# Autodesk Inventor assembly: Skateboard Box
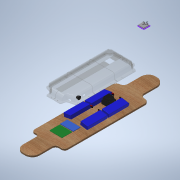
[picture p0: Inventor's stored thumbnail of the model, 180x180]
Saved by Autodesk Inventor 2020 (Build 240168000, 168)
## iProperties
Created: 2019-01-10
Part Number: Skateboard Box
Document SubType Name: Assembly
Designer: LSabe
Author: LSabe
## Documents named in this file (15)
- C:\Users\Luke\OneDrive\Desktop\Luke's stuff\Electric Skateboard\Electric_Skateboard V.2\Skateboard Files\Skateboard Box Files\Skateboard Box V2.iam
- C:\Users\Luke\OneDrive\Desktop\Luke's stuff\Electric Skateboard\Electric_Skateboard V.2\Skateboard Files\Skateboard Box Files\ESC.ipt
- C:\Users\LSabe\OneDrive\Documents\Inventor\Content Center Files\R2017\en-US\ANSI B18.6.3(03)\ANSI B18.6.3 - 10-32 UNF - 0.75(14).ipt
- C:\Users\Luke\OneDrive\Desktop\Luke's stuff\Electric Skateboard\Electric_Skateboard V.2\Skateboard Files\Skateboard Box Files\Battery.ipt
- C:\Users\Luke\OneDrive\Desktop\Luke's stuff\Electric Skateboard\Electric_Skateboard V.2\Skateboard Files\Skateboard Box Files\Lipo Charger Circuit.ipt
- C:\Users\Luke\OneDrive\Desktop\Luke's stuff\Electric Skateboard\Electric_Skateboard V.2\Skateboard Files\Skateboard Box Files\Receiver PCB.ipt
- C:\Users\Luke\OneDrive\Desktop\Luke's stuff\Electric Skateboard\Electric_Skateboard V.2\Skateboard Files\Skateboard Box Files\Power Switch.ipt
- C:\Users\Luke\OneDrive\Desktop\Luke's stuff\Electric Skateboard\Electric_Skateboard V.2\Skateboard Files\Skateboard Box Files\Skateboard Deck.ipt
- C:\Users\Luke\OneDrive\Desktop\Luke's stuff\Electric Skateboard\Electric_Skateboard V.2\Skateboard Files\Skateboard Box Files\Skateboard Box Back V2 a.ipt
- C:\Users\Luke\OneDrive\Desktop\Luke's stuff\Electric Skateboard\Electric_Skateboard V.2\Skateboard Files\Skateboard Box Files\Skateboard Box Back V2 b.ipt
- C:\Users\Luke\OneDrive\Desktop\Luke's stuff\Electric Skateboard\Electric_Skateboard V.2\Skateboard Files\Skateboard Box Files\Skateboard Box Front V2 a.ipt
- C:\Users\Luke\OneDrive\Desktop\Luke's stuff\Electric Skateboard\Electric_Skateboard V.2\Skateboard Files\Skateboard Box Files\Skateboard Box Front V2 b.ipt
- C:\Users\Luke\OneDrive\Desktop\Luke's stuff\Electric Skateboard\Electric_Skateboard V.2\Skateboard Files\Skateboard Box Files\Skateboard Box Middle V2 a.ipt
- C:\Users\Luke\OneDrive\Desktop\Luke's stuff\Electric Skateboard\Electric_Skateboard V.2\Skateboard Files\Skateboard Box Files\Skateboard Box Middle V2 b.ipt
- C:\Users\Luke\OneDrive\Desktop\Luke's stuff\Electric Skateboard\Electric_Skateboard V.2\Skateboard Files\Skateboard Box Files\Plug.ipt
## Components (34 placed, 14 different names)
1. ESC:1 — Mate:16, Mate:20
2. Receiver PCB:1 — Mate:15, Mate:17
3. Battery:1 — Mate:13, Flush:2, Flush:3
4. Battery:2 — Mate:14, Flush:2, Flush:4
5. Battery:3 — Mate:11, Flush:1, Flush:4
6. Battery:4 — Mate:12, Flush:1, Flush:3
7. Power Switch:1 — Mate:52, Mate:53
8. Skateboard Deck:1 — Mate:11, Mate:12, Mate:13, Mate:14, Mate:15, Mate:16, Mate:17, Mate:20, Mate:21, Mate:45, Mate:46, Flush:8, Flush:9, Mate:47, Mate:48, Flush:10, Mate:49
9. Lipo Charger Circuit:1 — Mate:21, Mate:45
10. Skateboard Box Back V2 a:1 — Flush:5, Flush:10, Flush:11, Flush:15, Mate:50, Mate:58, Mate:59, Mate:72, Mate:73
11. Skateboard Box Back V2 b:1 — Flush:5, Mate:48, Flush:11, Mate:64, Mate:65, Mate:68, Mate:69
12. Skateboard Box Front V2 a:1 — Flush:7, Flush:8, Flush:13, Flush:14, Mate:51, Mate:52, Mate:53, Mate:54, Mate:55, Mate:70, Mate:71
13. Skateboard Box Front V2 b:1 — Flush:7, Mate:46, Flush:13, Mate:60, Mate:61, Mate:66, Mate:67
14. Skateboard Box Middle V2 a:1 — Flush:6, Flush:9, Flush:12, Flush:14, Flush:15, Mate:50, Mate:51, Mate:56, Mate:57
15. Skateboard Box Middle V2 b:1 — Flush:6, Mate:47, Flush:12, Mate:49, Mate:62, Mate:63
16. Cross Recessed Binding Head Machine Screw - Type I - Inch No. 10 - 32 - 3/4:27 — Mate:66, Mate:67
17. Cross Recessed Binding Head Machine Screw - Type I - Inch No. 10 - 32 - 3/4:36 — Mate:70, Mate:71
18. Plug:1
19. Cross Recessed Binding Head Machine Screw - Type I - Inch No. 10 - 32 - 3/4:29 — Mate:60, Mate:61
20. Cross Recessed Binding Head Machine Screw - Type I - Inch No. 10 - 32 - 3/4:30
21. Cross Recessed Binding Head Machine Screw - Type I - Inch No. 10 - 32 - 3/4:26 — Mate:62, Mate:63
22. Cross Recessed Binding Head Machine Screw - Type I - Inch No. 10 - 32 - 3/4:31
23. Cross Recessed Binding Head Machine Screw - Type I - Inch No. 10 - 32 - 3/4:25 — Mate:64, Mate:65
24. Cross Recessed Binding Head Machine Screw - Type I - Inch No. 10 - 32 - 3/4:32
25. Cross Recessed Binding Head Machine Screw - Type I - Inch No. 10 - 32 - 3/4:22 — Mate:54, Mate:55
26. Cross Recessed Binding Head Machine Screw - Type I - Inch No. 10 - 32 - 3/4:33
27. Cross Recessed Binding Head Machine Screw - Type I - Inch No. 10 - 32 - 3/4:23 — Mate:56, Mate:57
28. Cross Recessed Binding Head Machine Screw - Type I - Inch No. 10 - 32 - 3/4:34
29. Cross Recessed Binding Head Machine Screw - Type I - Inch No. 10 - 32 - 3/4:24 — Mate:58, Mate:59
30. Cross Recessed Binding Head Machine Screw - Type I - Inch No. 10 - 32 - 3/4:35
31. Cross Recessed Binding Head Machine Screw - Type I - Inch No. 10 - 32 - 3/4:28 — Mate:68, Mate:69
32. Cross Recessed Binding Head Machine Screw - Type I - Inch No. 10 - 32 - 3/4:38
33. Cross Recessed Binding Head Machine Screw - Type I - Inch No. 10 - 32 - 3/4:37 — Mate:72, Mate:73
34. Cross Recessed Binding Head Machine Screw - Type I - Inch No. 10 - 32 - 3/4:39
## Component patterns: (2 elements, first: Cross Recessed Binding Head Machine Screw - Type I - Inch No. 10 - 32 - 3/4:29), (2 elements, first: Cross Recessed Binding Head Machine Screw - Type I - Inch No. 10 - 32 - 3/4:26), (2 elements, first: Cross Recessed Binding Head Machine Screw - Type I - Inch No. 10 - 32 - 3/4:25), (2 elements, first: Cross Recessed Binding Head Machine Screw - Type I - Inch No. 10 - 32 - 3/4:22), (2 elements, first: Cross Recessed Binding Head Machine Screw - Type I - Inch No. 10 - 32 - 3/4:23), (2 elements, first: Cross Recessed Binding Head Machine Screw - Type I - Inch No. 10 - 32 - 3/4:24), (2 elements, first: Cross Recessed Binding Head Machine Screw - Type I - Inch No. 10 - 32 - 3/4:28), (2 elements, first: Cross Recessed Binding Head Machine Screw - Type I - Inch No. 10 - 32 - 3/4:37)
## Relationships (53: Mate 38, Flush 15)
- Mate:11: Battery:3 ↔ Skateboard Deck:1
- Mate:12: Battery:4 ↔ Skateboard Deck:1
- Mate:13: Battery:1 ↔ Skateboard Deck:1
- Mate:14: Battery:2 ↔ Skateboard Deck:1
- Mate:15: Receiver PCB:1 ↔ Skateboard Deck:1
- Mate:16 (2.54 mm): ESC:1 ↔ Skateboard Deck:1
- Flush:1: Battery:3 ↔ Battery:4
- Flush:2: Battery:1 ↔ Battery:2
- Flush:3: Battery:1 ↔ Battery:4
- Flush:4: Battery:2 ↔ Battery:3
- Mate:17: Receiver PCB:1 ↔ Skateboard Deck:1
- Mate:20: ESC:1 ↔ Skateboard Deck:1
- Mate:21: Skateboard Deck:1 ↔ Lipo Charger Circuit:1
- Mate:45: Skateboard Deck:1 ↔ Lipo Charger Circuit:1
- Flush:5: Skateboard Box Back V2 a:1 ↔ Skateboard Box Back V2 b:1
- Flush:6: Skateboard Box Middle V2 a:1 ↔ Skateboard Box Middle V2 b:1
- Flush:7: Skateboard Box Front V2 a:1 ↔ Skateboard Box Front V2 b:1
- Mate:46: Skateboard Deck:1 ↔ Skateboard Box Front V2 b:1
- Flush:8: Skateboard Deck:1 ↔ Skateboard Box Front V2 a:1
- Flush:9: Skateboard Deck:1 ↔ Skateboard Box Middle V2 a:1
- Mate:47: Skateboard Deck:1 ↔ Skateboard Box Middle V2 b:1
- Mate:48: Skateboard Deck:1 ↔ Skateboard Box Back V2 b:1
- Flush:10: Skateboard Deck:1 ↔ Skateboard Box Back V2 a:1
- Flush:11: Skateboard Box Back V2 a:1 ↔ Skateboard Box Back V2 b:1
- Flush:12: Skateboard Box Middle V2 a:1 ↔ Skateboard Box Middle V2 b:1
- Flush:13: Skateboard Box Front V2 a:1 ↔ Skateboard Box Front V2 b:1
- Mate:49: Skateboard Deck:1 ↔ Skateboard Box Middle V2 b:1
- Flush:14: Skateboard Box Front V2 a:1 ↔ Skateboard Box Middle V2 a:1
- Flush:15: Skateboard Box Back V2 a:1 ↔ Skateboard Box Middle V2 a:1
- Mate:50: Skateboard Box Back V2 a:1 ↔ Skateboard Box Middle V2 a:1
- Mate:51: Skateboard Box Front V2 a:1 ↔ Skateboard Box Middle V2 a:1
- Mate:52: Power Switch:1 ↔ Skateboard Box Front V2 a:1
- Mate:53: Power Switch:1 ↔ Skateboard Box Front V2 a:1
- Mate:54: Skateboard Box Front V2 a:1 ↔ Cross Recessed Binding Head Machine Screw - Type I - Inch No. 10 - 32 - 3/4:22
- Mate:55: Skateboard Box Front V2 a:1 ↔ Cross Recessed Binding Head Machine Screw - Type I - Inch No. 10 - 32 - 3/4:22
- Mate:56: Skateboard Box Middle V2 a:1 ↔ Cross Recessed Binding Head Machine Screw - Type I - Inch No. 10 - 32 - 3/4:23
- Mate:57: Skateboard Box Middle V2 a:1 ↔ Cross Recessed Binding Head Machine Screw - Type I - Inch No. 10 - 32 - 3/4:23
- Mate:58: Skateboard Box Back V2 a:1 ↔ Cross Recessed Binding Head Machine Screw - Type I - Inch No. 10 - 32 - 3/4:24
- Mate:59: Skateboard Box Back V2 a:1 ↔ Cross Recessed Binding Head Machine Screw - Type I - Inch No. 10 - 32 - 3/4:24
- Mate:60: Skateboard Box Front V2 b:1 ↔ Cross Recessed Binding Head Machine Screw - Type I - Inch No. 10 - 32 - 3/4:29
- Mate:61: Skateboard Box Front V2 b:1 ↔ Cross Recessed Binding Head Machine Screw - Type I - Inch No. 10 - 32 - 3/4:29
- Mate:62: Skateboard Box Middle V2 b:1 ↔ Cross Recessed Binding Head Machine Screw - Type I - Inch No. 10 - 32 - 3/4:26
- Mate:63: Skateboard Box Middle V2 b:1 ↔ Cross Recessed Binding Head Machine Screw - Type I - Inch No. 10 - 32 - 3/4:26
- Mate:64: Skateboard Box Back V2 b:1 ↔ Cross Recessed Binding Head Machine Screw - Type I - Inch No. 10 - 32 - 3/4:25
- Mate:65: Skateboard Box Back V2 b:1 ↔ Cross Recessed Binding Head Machine Screw - Type I - Inch No. 10 - 32 - 3/4:25
- Mate:66: Skateboard Box Front V2 b:1 ↔ Cross Recessed Binding Head Machine Screw - Type I - Inch No. 10 - 32 - 3/4:27
- Mate:67: Skateboard Box Front V2 b:1 ↔ Cross Recessed Binding Head Machine Screw - Type I - Inch No. 10 - 32 - 3/4:27
- Mate:68: Skateboard Box Back V2 b:1 ↔ Cross Recessed Binding Head Machine Screw - Type I - Inch No. 10 - 32 - 3/4:28
- Mate:69: Skateboard Box Back V2 b:1 ↔ Cross Recessed Binding Head Machine Screw - Type I - Inch No. 10 - 32 - 3/4:28
- Mate:70: Skateboard Box Front V2 a:1 ↔ Cross Recessed Binding Head Machine Screw - Type I - Inch No. 10 - 32 - 3/4:36
- Mate:71: Skateboard Box Front V2 a:1 ↔ Cross Recessed Binding Head Machine Screw - Type I - Inch No. 10 - 32 - 3/4:36
- Mate:72: Skateboard Box Back V2 a:1 ↔ Cross Recessed Binding Head Machine Screw - Type I - Inch No. 10 - 32 - 3/4:37
- Mate:73: Skateboard Box Back V2 a:1 ↔ Cross Recessed Binding Head Machine Screw - Type I - Inch No. 10 - 32 - 3/4:37
